# Autodesk Inventor assembly: UBG-Antrieb_HR
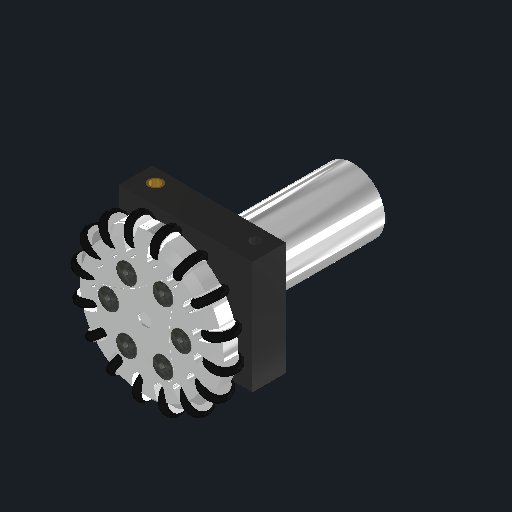
[picture p0: Inventor's stored thumbnail of the model, 512x512]
Saved by Autodesk Inventor 2025.2 (Build 292293000, 293)
## iProperties
Created: 2025-03-27
Part Number: UBG-Antrieb_HR
Document SubType Name: Assembly
Designer: Faabs
Author: Faabs
## Documents named in this file (6)
- C:\Users\Faabs\Desktop\TeamFaabs-CAD v2023\UBG\Antrieb\UBG-Antrieb_HR.iam
- C:\Users\Faabs\Desktop\TeamFaabs-CAD v2023\UBG\Antrieb\Motorhalterungen\Motorhalterung_HR.ipt
- C:\Users\Faabs\Desktop\TeamFaabs-CAD v2023\Verbindungselemente\Inventor\M3 Schmelzgewinde\M3 Schmelzgewinde\M3 Schmelzgewinde.ipt
- C:\Users\Faabs\Desktop\TeamFaabs-CAD v2023\UBG\Antrieb\Maxon DCX 19mm 13W\DCX 19mm 13W\DCX 19mm 13W\DCX 19mm 13W.ipt
- C:\Users\Faabs\Desktop\TeamFaabs-CAD v2023\Verbindungselemente\Inventor\ISO 7046\DIN EN ISO 7046-2 H - M2x6 - 8.8 - H1.ipt
- C:\Users\Faabs\Desktop\TeamFaabs-CAD v2023\UBG\Rad\UBG-Rad.iam
## Components (8 placed, 5 different names)
1. Motorhalterung_HR:1 — Passend:1, Passend:2, Passend:3, Passend:4, Fluchtend:1, Fluchtend:2, Fluchtend:3, Passend:5, Passend:6, Passend:7, Einfügen:1, Einfügen:2, Einfügen:3, Passend:9
2. DCX 19mm 13W:1 — Passend:5, Passend:6, Passend:7, Passend:8, Winkel:1
3. UBG-Rad:1 [sub-assembly] — Passend:8, Winkel:1, Passend:9
4. M3 Schmelzgewinde:1 — Passend:1, Fluchtend:3
5. M3 Schmelzgewinde:2 — Passend:2, Fluchtend:2
6. DIN EN ISO 7046-2 H M2x6 - 8.8 - H1:3 — Einfügen:3
7. DIN EN ISO 7046-2 H M2x6 - 8.8 - H1:2 — Einfügen:1
8. DIN EN ISO 7046-2 H M2x6 - 8.8 - H1:1 — Einfügen:2
## Relationships (16: Mate 9, Flush 3, Insert 3, Angle 1)
- Passend:1 [Mate]: Motorhalterung_HR:1 ↔ M3 Schmelzgewinde:1
- Passend:2 [Mate]: Motorhalterung_HR:1 ↔ M3 Schmelzgewinde:2
- Passend:3 [Mate]: Motorhalterung_HR:1
- Passend:4 [Mate]: Motorhalterung_HR:1
- Fluchtend:1 [Flush]: Motorhalterung_HR:1
- Fluchtend:2 [Flush] (0.1 mm): Motorhalterung_HR:1 ↔ M3 Schmelzgewinde:2
- Fluchtend:3 [Flush] (0.1 mm): Motorhalterung_HR:1 ↔ M3 Schmelzgewinde:1
- Passend:5 [Mate]: Motorhalterung_HR:1 ↔ DCX 19mm 13W:1
- Passend:6 [Mate]: Motorhalterung_HR:1 ↔ DCX 19mm 13W:1
- Passend:7 [Mate]: Motorhalterung_HR:1 ↔ DCX 19mm 13W:1
- Einfügen:1 [Insert]: Motorhalterung_HR:1 ↔ DIN EN ISO 7046-2 H M2x6 - 8.8 - H1:2
- Einfügen:2 [Insert]: Motorhalterung_HR:1 ↔ DIN EN ISO 7046-2 H M2x6 - 8.8 - H1:1
- Einfügen:3 [Insert]: Motorhalterung_HR:1 ↔ DIN EN ISO 7046-2 H M2x6 - 8.8 - H1:3
- Passend:8 [Mate]: DCX 19mm 13W:1 ↔ UBG-Rad:1
- Winkel:1 [Angle] (0 deg): DCX 19mm 13W:1 ↔ UBG-Rad:1
- Passend:9 [Mate] (0.1 mm): Motorhalterung_HR:1 ↔ UBG-Rad:1
